# Autodesk Inventor assembly: RotBase
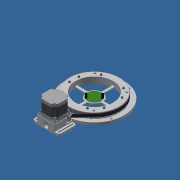
[picture p0: Inventor's stored thumbnail of the model, 180x180]
Saved by Autodesk Inventor 2016 (Build 200138000, 138)
## iProperties
Created: 2015-10-03
Part Number: RotBase
Material: Generisch
Document SubType Name: Assembly
Designer: 4ndreas
Mass: 1429.37 g
Surface Area: 3754.16 cm^2
Volume: 1275.86 cm^3
Density: 1.12032 g/cm^3
Author: 4ndreas
## Documents named in this file (21)
- C:\Users\4ndreas\Documents\Inventor\RobotARM v2\v4\_assemblys\RotBase.iam
- C:\Users\4ndreas\Documents\Inventor\RobotARM v2\v4\_printed parts\RotBase.ipt
- C:\Users\4ndreas\Documents\Inventor\RobotARM v2\v4\RotBase\Konstruktions-Assistent\Übertragung des Zahnriemens1.iam
- C:\Users\4ndreas\Documents\Inventor\RobotARM v2\v4\_misc parts\Drehkranz.ipt
- C:\Users\4ndreas\Documents\Inventor\RobotARM v2\v4\_encoder\encoder_bare.ipt
- C:\Users\4ndreas\Documents\Inventor\Content Center Files\R2014\de-DE\DIN 9021\DIN 9021 - 4,3.ipt
- C:\Users\4ndreas\Documents\Inventor\Content Center Files\R2014\de-DE\DIN 125-1  A\DIN 125 - A 4,3.ipt
- C:\Users\4ndreas\Documents\Inventor\RobotARM v2\v4\_standard Parts\DIN 625 SKF - SKF 624_flansch.ipt
- C:\Users\4ndreas\Documents\Inventor\Content Center Files\R2014\de-DE\DIN BEARING(1)\DIN 625 SKF - SKF 624.ipt
- C:\Users\4ndreas\Documents\Inventor\RobotARM v2\v4\_metal parts\16221600.ipt
- C:\Users\4ndreas\Documents\Inventor\Content Center Files\R2014\de-DE\DIN 125-1  A\DIN 125 - A 5,3.ipt
- C:\Users\4ndreas\Documents\Inventor\Content Center Files\R2014\de-DE\DIN 934\DIN 934 - M4 x 0,7.ipt
- C:\Users\4ndreas\Documents\Inventor\RobotARM v2\v4\_printed parts\rotBaseMagnetMount.ipt
- C:\Users\4ndreas\Documents\Inventor\RobotARM v2\v4\_encoder\EncoderMagnet.ipt
- C:\Users\4ndreas\Documents\Inventor\Content Center Files\R2014\de-DE\DIN 7991(2)\DIN 7991 - M4x25.ipt
- C:\Users\4ndreas\Documents\Inventor\Content Center Files\R2014\de-DE\DIN 7991(2)\DIN 7991 - M4x30.ipt
- C:\Users\4ndreas\Documents\Inventor\RobotARM v2\v4\_printed parts\rotNema23Mount.ipt
- C:\Users\4ndreas\Documents\Inventor\Content Center Files\R2014\de-DE\DIN 933\DIN 933 - M4  x 40.ipt
- C:\Users\4ndreas\Documents\Inventor\RobotARM v2\v4\_misc parts\Drehkranz_B.ipt
- C:\Users\4ndreas\Documents\Inventor\Content Center Files\R2014\de-DE\DIN 913\DIN 913 - M4 x 4.ipt
- C:\Users\4ndreas\Documents\Inventor\RobotARM v2\v4\_motors\Nema23.ipt
## Components (51 placed, 20 different names)
1. Übertragung des Zahnriemens:1 [sub-assembly] — Passend:2, Passend:7, Passend:15
2. Nema23:1 — Passend:2, Winkel:1, Winkel:2, Passend:51, Passend:52, Passend:53, Einfügen:9, Einfügen:10, Einfügen:11, Einfügen:12
3. Drehkranz:1 — Passend:3, Passend:4, Passend:5, Fluchtend:1, Fluchtend:2, Passend:66, Passend:67, Fluchtend:3, Fluchtend:4, Passend:69, Passend:70, Fluchtend:5, Fluchtend:6, Fluchtend:15, Passend:101
4. RotBase:1 — Passend:5, Passend:6, Passend:16, Passend:17, Passend:68, Passend:75, Passend:76, Passend:77, Passend:78, Passend:79, Passend:80, Passend:81, Passend:82, Passend:83, Fluchtend:7, Passend:84, Passend:85, Passend:86, Passend:87, Passend:88, Passend:89, Passend:90, Fluchtend:8, Fluchtend:9, Fluchtend:10, Fluchtend:11, Fluchtend:12, Fluchtend:13, Fluchtend:14
5. encoder_bare:1 — Passend:15, Passend:16, Passend:17
6. rotNema23Mount:1 — Fluchtend:1, Winkel:1, Passend:19, Passend:21, Passend:22, Passend:41, Passend:42, Passend:53, Passend:62, Passend:91, Passend:92, Passend:93, Passend:94, Passend:95, Passend:96
7. DIN 933 - ersetzt durch DIN EN 24017 M4  x 40:3 — Passend:21, Passend:23, Passend:24, Passend:43, Passend:48, Passend:55, Passend:62
8. DIN 933 - ersetzt durch DIN EN 24017 M4  x 40:4 — Passend:19, Passend:22, Passend:25, Passend:26, Passend:44, Passend:45, Passend:54
9. DIN 9021 4,3:1 — Einfügen:4, Passend:41, Passend:44
10. DIN 9021 4,3:2 — Einfügen:3, Passend:42, Passend:43
11. DIN 125-1 A A 4,3:1 — Einfügen:3, Passend:28
12. DIN 125-1 A A 4,3:2 — Einfügen:4, Passend:27
13. F624 ZZ 4x13x5:1 — Passend:25, Einfügen:7, Passend:46
14. F624 ZZ 4x13x5:2 — Passend:24, Passend:28, Passend:50
15. F624 ZZ 4x13x5:3 — Passend:23, Einfügen:8, Passend:49
16. F624 ZZ 4x13x5:4 — Passend:26, Passend:27, Passend:47
17. DIN 125-1 A A 4,3:5 — Einfügen:7
18. DIN 125-1 A A 4,3:6 — Einfügen:8
19. DIN 625 SKF SKF 624:1 — Passend:48, Passend:49, Passend:50
20. DIN 625 SKF SKF 624:2 — Passend:45, Passend:46, Passend:47
21. 16221600:1 — Passend:51, Passend:52, Passend:102
22. DIN 125-1 A A 5,3:1 — Einfügen:9, Passend:57
23. DIN 125-1 A A 5,3:2 — Einfügen:10, Passend:100
24. DIN 125-1 A A 5,3:3 — Einfügen:11, Passend:56
25. DIN 125-1 A A 5,3:4 — Einfügen:12, Passend:99
26. DIN 934 - ersetzt durch DIN EN 24032/28673/28674 M4:1 — Passend:55, Passend:56
27. DIN 934 - ersetzt durch DIN EN 24032/28673/28674 M4:2 — Passend:54, Passend:57
28. rotBaseMagnetMount:1 — Passend:63, Passend:64, Passend:65, Fluchtend:2
29. EncoderMagnet:1 — Passend:63, Passend:64
30. DIN 7991 M4x30:1 — Passend:66, Fluchtend:4, Passend:71
31. DIN 7991 M4x30:2 — Passend:67, Passend:68, Fluchtend:3, Passend:72
32. DIN 7991 M4x30:3 — Passend:69, Fluchtend:5, Passend:73
33. DIN 7991 M4x30:4 — Passend:70, Fluchtend:6, Passend:74
34. DIN 934 - ersetzt durch DIN EN 24032/28673/28674 M4:3 — Passend:74, Passend:78, Passend:79
35. DIN 934 - ersetzt durch DIN EN 24032/28673/28674 M4:4 — Passend:73, Passend:77, Passend:80
36. DIN 934 - ersetzt durch DIN EN 24032/28673/28674 M4:5 — Passend:72, Passend:76, Passend:81
37. DIN 934 - ersetzt durch DIN EN 24032/28673/28674 M4:6 — Passend:71, Passend:75, Passend:82
38. DIN 7991 M4x25:1 — Passend:83, Fluchtend:7
39. DIN 7991 M4x25:2 — Passend:85, Fluchtend:14
40. DIN 7991 M4x25:3 — Passend:87, Fluchtend:12
41. DIN 7991 M4x25:4 — Passend:88, Fluchtend:8
42. DIN 7991 M4x25:5 — Passend:86, Fluchtend:13
43. DIN 7991 M4x25:6 — Passend:84, Fluchtend:9
44. DIN 7991 M4x25:7 — Passend:89, Fluchtend:10
45. DIN 7991 M4x25:8 — Passend:90, Fluchtend:11
46. DIN 933 - ersetzt durch DIN EN 24017 M4  x 40:1 — Passend:91, Passend:93, Passend:96, Passend:97
47. DIN 933 - ersetzt durch DIN EN 24017 M4  x 40:2 — Passend:92, Passend:94, Passend:95, Passend:98
48. DIN 934 - ersetzt durch DIN EN 24032/28673/28674 M4:7 — Passend:97, Passend:99
49. DIN 934 - ersetzt durch DIN EN 24032/28673/28674 M4:8 — Passend:98, Passend:100
50. Drehkranz_B:1 — Fluchtend:15, Passend:101
51. DIN 913 M4 x 4:1 — Passend:102
## Relationships (101: Mate 76, Flush 15, Insert 8, Angle 2)
- Passend:2 [Mate]: Übertragung des Zahnriemens:1 ↔ Nema23:1
- Passend:3 [Mate]: Drehkranz:1
- Passend:4 [Mate]: Drehkranz:1
- Passend:5 [Mate]: Drehkranz:1 ↔ RotBase:1
- Passend:6 [Mate]: RotBase:1
- Passend:7 [Mate]: Übertragung des Zahnriemens:1
- Passend:15 [Mate]: Übertragung des Zahnriemens:1 ↔ encoder_bare:1
- Passend:16 [Mate]: RotBase:1 ↔ encoder_bare:1
- Passend:17 [Mate]: RotBase:1 ↔ encoder_bare:1
- Fluchtend:1 [Flush]: Drehkranz:1 ↔ rotNema23Mount:1
- Winkel:1 [Angle] (0 deg): Nema23:1 ↔ rotNema23Mount:1
- Winkel:2 [Angle] (-90 deg): Nema23:1
- Passend:19 [Mate]: rotNema23Mount:1 ↔ DIN 933 - ersetzt durch DIN EN 24017 M4  x 40:4
- Passend:21 [Mate]: rotNema23Mount:1 ↔ DIN 933 - ersetzt durch DIN EN 24017 M4  x 40:3
- Passend:22 [Mate]: rotNema23Mount:1 ↔ DIN 933 - ersetzt durch DIN EN 24017 M4  x 40:4
- Einfügen:3 [Insert]: DIN 9021 4,3:2 ↔ DIN 125-1 A A 4,3:1
- Einfügen:4 [Insert]: DIN 9021 4,3:1 ↔ DIN 125-1 A A 4,3:2
- Passend:23 [Mate]: DIN 933 - ersetzt durch DIN EN 24017 M4  x 40:3 ↔ F624 ZZ 4x13x5:3
- Passend:24 [Mate]: DIN 933 - ersetzt durch DIN EN 24017 M4  x 40:3 ↔ F624 ZZ 4x13x5:2
- Passend:25 [Mate]: DIN 933 - ersetzt durch DIN EN 24017 M4  x 40:4 ↔ F624 ZZ 4x13x5:1
- Passend:26 [Mate]: DIN 933 - ersetzt durch DIN EN 24017 M4  x 40:4 ↔ F624 ZZ 4x13x5:4
- Passend:27 [Mate]: DIN 125-1 A A 4,3:2 ↔ F624 ZZ 4x13x5:4
- Passend:28 [Mate]: DIN 125-1 A A 4,3:1 ↔ F624 ZZ 4x13x5:2
- Einfügen:7 [Insert]: F624 ZZ 4x13x5:1 ↔ DIN 125-1 A A 4,3:5
- Einfügen:8 [Insert]: F624 ZZ 4x13x5:3 ↔ DIN 125-1 A A 4,3:6
- Passend:41 [Mate]: rotNema23Mount:1 ↔ DIN 9021 4,3:1
- Passend:42 [Mate]: rotNema23Mount:1 ↔ DIN 9021 4,3:2
- Passend:43 [Mate]: DIN 933 - ersetzt durch DIN EN 24017 M4  x 40:3 ↔ DIN 9021 4,3:2
- Passend:44 [Mate]: DIN 933 - ersetzt durch DIN EN 24017 M4  x 40:4 ↔ DIN 9021 4,3:1
- Passend:45 [Mate]: DIN 933 - ersetzt durch DIN EN 24017 M4  x 40:4 ↔ DIN 625 SKF SKF 624:2
- Passend:46 [Mate]: F624 ZZ 4x13x5:1 ↔ DIN 625 SKF SKF 624:2
- Passend:47 [Mate]: F624 ZZ 4x13x5:4 ↔ DIN 625 SKF SKF 624:2
- Passend:48 [Mate]: DIN 933 - ersetzt durch DIN EN 24017 M4  x 40:3 ↔ DIN 625 SKF SKF 624:1
- Passend:49 [Mate]: F624 ZZ 4x13x5:3 ↔ DIN 625 SKF SKF 624:1
- Passend:50 [Mate]: F624 ZZ 4x13x5:2 ↔ DIN 625 SKF SKF 624:1
- Passend:51 [Mate]: Nema23:1 ↔ 16221600:1
- Passend:52 [Mate] (0.2 mm): Nema23:1 ↔ 16221600:1
- Passend:53 [Mate]: Nema23:1 ↔ rotNema23Mount:1
- Einfügen:9 [Insert]: Nema23:1 ↔ DIN 125-1 A A 5,3:1
- Einfügen:10 [Insert]: Nema23:1 ↔ DIN 125-1 A A 5,3:2
- Einfügen:11 [Insert]: Nema23:1 ↔ DIN 125-1 A A 5,3:3
- Einfügen:12 [Insert]: Nema23:1 ↔ DIN 125-1 A A 5,3:4
- Passend:54 [Mate]: DIN 933 - ersetzt durch DIN EN 24017 M4  x 40:4 ↔ DIN 934 - ersetzt durch DIN EN 24032/28673/28674 M4:2
- Passend:55 [Mate]: DIN 933 - ersetzt durch DIN EN 24017 M4  x 40:3 ↔ DIN 934 - ersetzt durch DIN EN 24032/28673/28674 M4:1
- Passend:56 [Mate]: DIN 125-1 A A 5,3:3 ↔ DIN 934 - ersetzt durch DIN EN 24032/28673/28674 M4:1
- Passend:57 [Mate]: DIN 125-1 A A 5,3:1 ↔ DIN 934 - ersetzt durch DIN EN 24032/28673/28674 M4:2
- Passend:62 [Mate]: rotNema23Mount:1 ↔ DIN 933 - ersetzt durch DIN EN 24017 M4  x 40:3
- Passend:63 [Mate]: rotBaseMagnetMount:1 ↔ EncoderMagnet:1
- Passend:64 [Mate]: rotBaseMagnetMount:1 ↔ EncoderMagnet:1
- Passend:65 [Mate]: rotBaseMagnetMount:1
- Fluchtend:2 [Flush]: Drehkranz:1 ↔ rotBaseMagnetMount:1
- Passend:66 [Mate]: Drehkranz:1 ↔ DIN 7991 M4x30:1
- Passend:67 [Mate]: Drehkranz:1 ↔ DIN 7991 M4x30:2
- Passend:68 [Mate]: RotBase:1 ↔ DIN 7991 M4x30:2
- Fluchtend:3 [Flush]: Drehkranz:1 ↔ DIN 7991 M4x30:2
- Fluchtend:4 [Flush]: Drehkranz:1 ↔ DIN 7991 M4x30:1
- Passend:69 [Mate]: Drehkranz:1 ↔ DIN 7991 M4x30:3
- Passend:70 [Mate]: Drehkranz:1 ↔ DIN 7991 M4x30:4
- Fluchtend:5 [Flush]: Drehkranz:1 ↔ DIN 7991 M4x30:3
- Fluchtend:6 [Flush]: Drehkranz:1 ↔ DIN 7991 M4x30:4
- Passend:71 [Mate]: DIN 7991 M4x30:1 ↔ DIN 934 - ersetzt durch DIN EN 24032/28673/28674 M4:6
- Passend:72 [Mate]: DIN 7991 M4x30:2 ↔ DIN 934 - ersetzt durch DIN EN 24032/28673/28674 M4:5
- Passend:73 [Mate]: DIN 7991 M4x30:3 ↔ DIN 934 - ersetzt durch DIN EN 24032/28673/28674 M4:4
- Passend:74 [Mate]: DIN 7991 M4x30:4 ↔ DIN 934 - ersetzt durch DIN EN 24032/28673/28674 M4:3
- Passend:75 [Mate]: RotBase:1 ↔ DIN 934 - ersetzt durch DIN EN 24032/28673/28674 M4:6
- Passend:76 [Mate]: RotBase:1 ↔ DIN 934 - ersetzt durch DIN EN 24032/28673/28674 M4:5
- Passend:77 [Mate]: RotBase:1 ↔ DIN 934 - ersetzt durch DIN EN 24032/28673/28674 M4:4
- Passend:78 [Mate]: RotBase:1 ↔ DIN 934 - ersetzt durch DIN EN 24032/28673/28674 M4:3
- Passend:79 [Mate]: RotBase:1 ↔ DIN 934 - ersetzt durch DIN EN 24032/28673/28674 M4:3
- Passend:80 [Mate]: RotBase:1 ↔ DIN 934 - ersetzt durch DIN EN 24032/28673/28674 M4:4
- Passend:81 [Mate]: RotBase:1 ↔ DIN 934 - ersetzt durch DIN EN 24032/28673/28674 M4:5
- Passend:82 [Mate]: RotBase:1 ↔ DIN 934 - ersetzt durch DIN EN 24032/28673/28674 M4:6
- Passend:83 [Mate]: RotBase:1 ↔ DIN 7991 M4x25:1
- Fluchtend:7 [Flush]: RotBase:1 ↔ DIN 7991 M4x25:1
- Passend:84 [Mate]: RotBase:1 ↔ DIN 7991 M4x25:6
- Passend:85 [Mate]: RotBase:1 ↔ DIN 7991 M4x25:2
- Passend:86 [Mate]: RotBase:1 ↔ DIN 7991 M4x25:5
- Passend:87 [Mate]: RotBase:1 ↔ DIN 7991 M4x25:3
- Passend:88 [Mate]: RotBase:1 ↔ DIN 7991 M4x25:4
- Passend:89 [Mate]: RotBase:1 ↔ DIN 7991 M4x25:7
- Passend:90 [Mate]: RotBase:1 ↔ DIN 7991 M4x25:8
- Fluchtend:8 [Flush]: RotBase:1 ↔ DIN 7991 M4x25:4
- Fluchtend:9 [Flush]: RotBase:1 ↔ DIN 7991 M4x25:6
- Fluchtend:10 [Flush]: RotBase:1 ↔ DIN 7991 M4x25:7
- Fluchtend:11 [Flush]: RotBase:1 ↔ DIN 7991 M4x25:8
- Fluchtend:12 [Flush]: RotBase:1 ↔ DIN 7991 M4x25:3
- Fluchtend:13 [Flush]: RotBase:1 ↔ DIN 7991 M4x25:5
- Fluchtend:14 [Flush]: RotBase:1 ↔ DIN 7991 M4x25:2
- Passend:91 [Mate]: rotNema23Mount:1 ↔ DIN 933 - ersetzt durch DIN EN 24017 M4  x 40:1
- Passend:92 [Mate]: rotNema23Mount:1 ↔ DIN 933 - ersetzt durch DIN EN 24017 M4  x 40:2
- Passend:93 [Mate]: rotNema23Mount:1 ↔ DIN 933 - ersetzt durch DIN EN 24017 M4  x 40:1
- Passend:94 [Mate]: rotNema23Mount:1 ↔ DIN 933 - ersetzt durch DIN EN 24017 M4  x 40:2
- Passend:95 [Mate]: rotNema23Mount:1 ↔ DIN 933 - ersetzt durch DIN EN 24017 M4  x 40:2
- Passend:96 [Mate]: rotNema23Mount:1 ↔ DIN 933 - ersetzt durch DIN EN 24017 M4  x 40:1
- Passend:97 [Mate]: DIN 933 - ersetzt durch DIN EN 24017 M4  x 40:1 ↔ DIN 934 - ersetzt durch DIN EN 24032/28673/28674 M4:7
- Passend:98 [Mate]: DIN 933 - ersetzt durch DIN EN 24017 M4  x 40:2 ↔ DIN 934 - ersetzt durch DIN EN 24032/28673/28674 M4:8
- Passend:99 [Mate]: DIN 125-1 A A 5,3:4 ↔ DIN 934 - ersetzt durch DIN EN 24032/28673/28674 M4:7
- Passend:100 [Mate]: DIN 125-1 A A 5,3:2 ↔ DIN 934 - ersetzt durch DIN EN 24032/28673/28674 M4:8
- Fluchtend:15 [Flush]: Drehkranz:1 ↔ Drehkranz_B:1
- Passend:101 [Mate]: Drehkranz:1 ↔ Drehkranz_B:1
- Passend:102 [Mate]: 16221600:1 ↔ DIN 913 M4 x 4:1
